# Autodesk Inventor assembly: MainAssembly
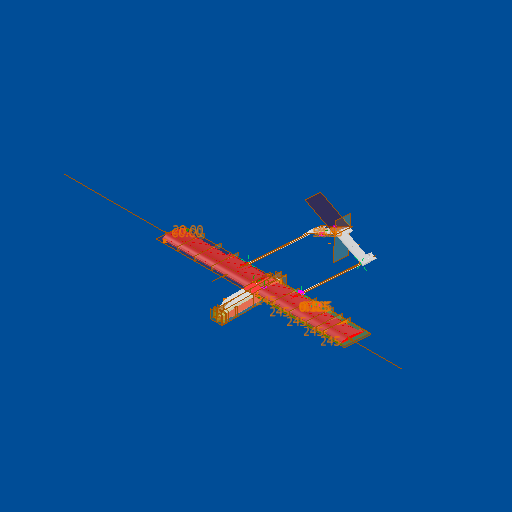
[picture p0: Inventor's stored thumbnail of the model, 512x512]
Saved by Autodesk Inventor 2027.1 (Build 311270010, 270A)
## iProperties
Created: 2026-09-14
Part Number: MainAssembly
Document SubType Name: Assembly
Designer: mateo
Author: mateo
## Documents named in this file (10)
- C:\GitHub\SWIFT-UAV\System_development\Pelican\structural_model\v0.3.1\MainAssembly\MainAssembly.iam
- C:\GitHub\SWIFT-UAV\System_development\Pelican\structural_model\v0.3.1\Parts\Aluminum_20x20\20x20x1295ExtrudedAluminum_MIR1.ipt
- C:\GitHub\SWIFT-UAV\System_development\Pelican\structural_model\v0.3.1\Parts\Fuselage\FuselageV3.ipt
- C:\GitHub\SWIFT-UAV\System_development\Pelican\structural_model\v0.3.1\Parts\Wings\WingBox_v2.ipt
- C:\GitHub\SWIFT-UAV\System_development\Pelican\structural_model\v0.3.1\Parts\Ancillary Components\MotorHousingV3.ipt
- C:\GitHub\SWIFT-UAV\System_development\Pelican\structural_model\v0.3.1\Parts\Wings\WingLeft_v0.1_MIR.ipt
- C:\GitHub\SWIFT-UAV\System_development\Pelican\structural_model\v0.3.1\Parts\Wings\WingLeft_v0.1.ipt
- C:\GitHub\SWIFT-UAV\System_development\Pelican\structural_model\v0.3.1\Parts\Cover\FrontCover.ipt
- C:\GitHub\SWIFT-UAV\System_development\Pelican\structural_model\v0.3.1\Parts\Delb_Parts\NewTail(final).iam
- C:\GitHub\SWIFT-UAV\System_development\Pelican\structural_model\v0.3.1\Parts\Aluminum_20x20\20x20x800ExtrudedAluminum_MIR.ipt
## Components (11 placed, 9 different names)
1. FuselageV3:1 — Mate:1, Mate:2, Mate:3, Mate:4, Mate:5, Mate:6, Mate:7, Mate:16, Mate:17, Mate:36
2. WingBox_v2:1 — Mate:4, Mate:5, Mate:18, Mate:19, Mate:20, Mate:21, Mate:22, Mate:26, Mate:29
3. MotorHousingV3:1 — Mate:6, Mate:7
4. FrontCover:1 — Mate:15, Mate:16, Mate:17
5. 20x20x1295ExtrudedAluminum_MIR1:1 — Mate:18, Mate:19, Mate:20, Mate:23, Mate:24, Mate:25
6. 20x20x1295ExtrudedAluminum_MIR1:2 — Mate:21, Mate:22, Mate:23, Mate:27, Mate:28
7. NewTail(final):1 [sub-assembly] — Mate:30, Mate:31, Mate:34, Mate:35, Mate:36, Mate:37
8. WingLeft_v0.1:1 — Mate:24, Mate:25, Mate:26, Mate:38, Mate:39
9. WingLeft_v0.1_MIR:1 — Mate:27, Mate:28, Mate:29
10. 20x20x800ExtrudedAluminum_MIR:1 — Mate:30, Mate:31, Mate:34
11. 20x20x800ExtrudedAluminum_MIR:2 — Mate:35, Mate:37, Mate:38, Mate:39
## Relationships (30: Mate 30)
- Mate:1: FuselageV3:1
- Mate:2: FuselageV3:1
- Mate:3: FuselageV3:1
- Mate:4: FuselageV3:1 ↔ WingBox_v2:1
- Mate:5: FuselageV3:1 ↔ WingBox_v2:1
- Mate:6: FuselageV3:1 ↔ MotorHousingV3:1
- Mate:7: FuselageV3:1 ↔ MotorHousingV3:1
- Mate:15: FrontCover:1
- Mate:16: FuselageV3:1 ↔ FrontCover:1
- Mate:17: FuselageV3:1 ↔ FrontCover:1
- Mate:18 (0.134 mm): WingBox_v2:1 ↔ 20x20x1295ExtrudedAluminum_MIR1:1
- Mate:19 (0.12 mm): WingBox_v2:1 ↔ 20x20x1295ExtrudedAluminum_MIR1:1
- Mate:20 (0.2 mm): WingBox_v2:1 ↔ 20x20x1295ExtrudedAluminum_MIR1:1
- Mate:21 (0.12 mm): WingBox_v2:1 ↔ 20x20x1295ExtrudedAluminum_MIR1:2
- Mate:22 (0.134 mm): WingBox_v2:1 ↔ 20x20x1295ExtrudedAluminum_MIR1:2
- Mate:23 (0.2 mm): 20x20x1295ExtrudedAluminum_MIR1:1 ↔ 20x20x1295ExtrudedAluminum_MIR1:2
- Mate:24 (0.125 mm): 20x20x1295ExtrudedAluminum_MIR1:1 ↔ WingLeft_v0.1:1
- Mate:25 (0.125 mm): 20x20x1295ExtrudedAluminum_MIR1:1 ↔ WingLeft_v0.1:1
- Mate:26 (0.2 mm): WingBox_v2:1 ↔ WingLeft_v0.1:1
- Mate:27 (0.125 mm): 20x20x1295ExtrudedAluminum_MIR1:2 ↔ WingLeft_v0.1_MIR:1
- Mate:28 (0.125 mm): 20x20x1295ExtrudedAluminum_MIR1:2 ↔ WingLeft_v0.1_MIR:1
- Mate:29 (0.2 mm): WingBox_v2:1 ↔ WingLeft_v0.1_MIR:1
- Mate:30 (0.25 mm): NewTail(final):1 ↔ 20x20x800ExtrudedAluminum_MIR:1
- Mate:31 (0.25 mm): NewTail(final):1 ↔ 20x20x800ExtrudedAluminum_MIR:1
- Mate:34: NewTail(final):1 ↔ 20x20x800ExtrudedAluminum_MIR:1
- Mate:35: NewTail(final):1 ↔ 20x20x800ExtrudedAluminum_MIR:2
- Mate:36: FuselageV3:1 ↔ NewTail(final):1
- Mate:37 (0.125 mm): NewTail(final):1 ↔ 20x20x800ExtrudedAluminum_MIR:2
- Mate:38 (0.125 mm): WingLeft_v0.1:1 ↔ 20x20x800ExtrudedAluminum_MIR:2
- Mate:39: WingLeft_v0.1:1 ↔ 20x20x800ExtrudedAluminum_MIR:2
